# Autodesk Inventor assembly: Hudson 1-69
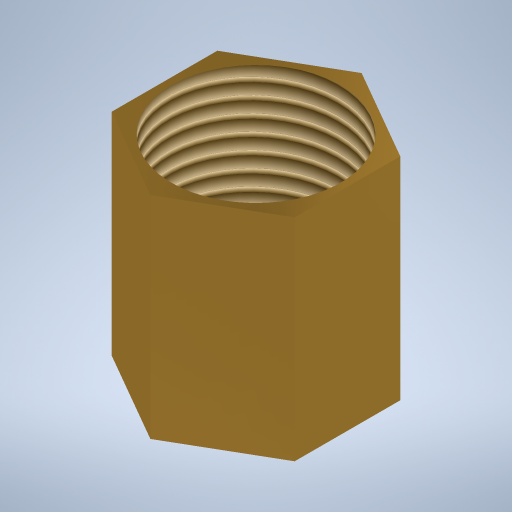
[picture p0: Inventor's stored thumbnail of the model, 512x512]
Saved by Autodesk Inventor 2024.2 (Build 282272000, 272)
## iProperties
Created: 2024-11-02
Part Number: Hudson 1-69
Document SubType Name: Assembly
Designer: Monica Mora
Author: Monica Mora
## Documents named in this file (3)
- C:\Users\Monica Mora\Desktop\Proyecto Locomotora\Hudson 1-69.iam
- C:\Users\Monica Mora\Desktop\Proyecto Locomotora\Pieza 1 subensamble 1-69.ipt
- C:\Users\Monica Mora\Desktop\Proyecto Locomotora\Pieza 2 subensamble 1-69.ipt
## Components (2 placed, 2 different names)
1. Pieza 1 subensamble 1-69:1 — Coincidencia:1, Coincidencia:2
2. Pieza 2 subensamble 1-69:1 — Coincidencia:1, Coincidencia:2
## Relationships (2: Mate 2)
- Coincidencia:1 [Mate]: Pieza 1 subensamble 1-69:1 ↔ Pieza 2 subensamble 1-69:1
- Coincidencia:2 [Mate]: Pieza 1 subensamble 1-69:1 ↔ Pieza 2 subensamble 1-69:1
